# Autodesk Inventor assembly: BHSS
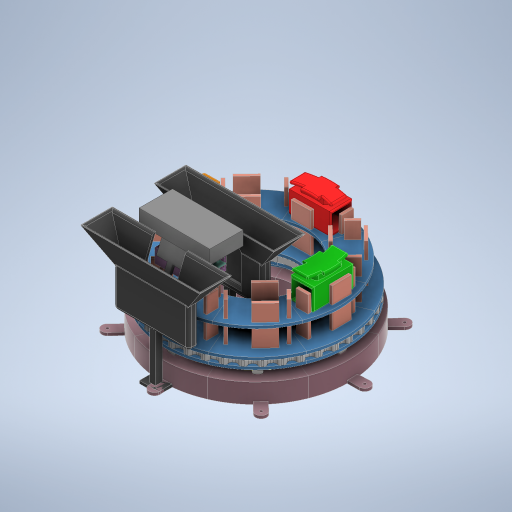
[picture p0: Inventor's stored thumbnail of the model, 512x512]
Saved by Autodesk Inventor 2023 (Build 270158000, 158)
## iProperties
Created: 2022-10-26
Part Number: BHSS
Document SubType Name: Assembly
Designer: cheng
Mass: 107138 g
Surface Area: 105016 cm^2
Volume: 89092.4 cm^3
Density: 1.20255 g/cm^3
Author: cheng
## Documents named in this file (11)
- C:\Users\mihal\Desktop\Current BHSS Design\Eighth Assembly\BHSS.iam
- C:\Users\mihal\Desktop\Current BHSS Design\Eighth Assembly\Battery Container.ipt
- C:\Users\mihal\Desktop\Current BHSS Design\Eighth Assembly\Box Base Plate.ipt
- C:\Users\mihal\Desktop\Current BHSS Design\Eighth Assembly\Carousel Fixed Track.ipt
- C:\Users\mihal\Desktop\Current BHSS Design\Eighth Assembly\drone model.ipt
- C:\Users\mihal\Desktop\Current BHSS Design\Eighth Assembly\Husky_3D_Model.ipt
- C:\Users\mihal\Desktop\Current BHSS Design\Eighth Assembly\Landing dock V2.ipt
- C:\Users\mihal\Desktop\Current BHSS Design\Eighth Assembly\Battery Cage Spring Plate.ipt
- C:\Users\mihal\Desktop\Current BHSS Design\Eighth Assembly\Inner Circle Landing Legs.ipt
- C:\Users\mihal\Desktop\Current BHSS Design\Eighth Assembly\Full Roller Carousel Assembly.iam
- C:\Users\mihal\Desktop\Current BHSS Design\Eighth Assembly\Battery Cage - Copy.ipt
## Components (25 placed, 13 different names)
1. Box Base Plate:1 — Mate:4, Mate:5, Mate:6, Mate:18, Mate:19, Mate:20, Mate:25, Flush:1, Mate:107, Mate:110, Mate:111, Mate:117, Mate:118
2. Carousel Fixed Track:1 — Mate:4, Mate:10, Mate:11
3. Carousel Fixed Track:2 — Mate:5, Mate:14, Mate:15, Mate:16, Mate:17, Mate:119
4. Carousel Fixed Track:3 — Mate:10, Mate:11, Mate:12, Mate:13, Mate:25, Rotating the Crousel
5. Carousel Fixed Track:4 — Mate:6, Mate:12, Mate:13, Mate:14, Mate:15, Mate:120
6. Carousel Fixed Track:5 — Mate:16, Mate:17, Mate:18, Mate:21, Mate:22
7. Carousel Fixed Track:6 — Mate:19, Mate:23, Mate:24, Mate:108, Mate:109
8. Carousel Fixed Track:7 — Mate:20, Mate:21, Mate:22, Mate:23, Mate:24
9. drone model:1 — Mate:145, Mate:146, Mate:147
10. Husky_3D_Model:1 — Flush:1
11. Red Battery — Side, Front, Bottom, Bat Wing Face to Cage Face, Mate:152
12. Carousel Fixed Track:8 — Mate:107, Mate:108, Mate:109
13. Landing dock V2:1 — Mate:110, Mate:111
14. Battery Cage Spring Plate:2 — Mate:148, Spring and top, Mate:152, Mate:153
15. Inner Circle Landing Legs:2 — Mate:117
16. Inner Circle Landing Legs:4 — Mate:118
17. Full Roller Carousel Assembly:1 [sub-assembly] — Mate:119, Mate:120, Side, Front, Mate:123, Mate:124, Mate:125, Mate:126, Mate:127, Mate:128, Mate:129, Mate:130, Mate:131, Mate:132, Mate:133, Mate:134, Mate:135, Mate:136, Mate:137, Mate:138, Mate:139, Mate:140, Mate:141, Mate:142, Bottom, Mate:144, Rotating the Crousel
18. Battery Container:20 — Mate:127, Mate:128, Mate:140
19. Battery Container:21 — Mate:131, Mate:132, Mate:138
20. Green Battery — Mate:125, Mate:126, Mate:141, Mate:153
21. Battery Container:23 — Mate:129, Mate:130, Mate:139
22. Orange Battery — Mate:133, Mate:134, Mate:137
23. Battery Container:25 — Mate:135, Mate:136, Mate:144
24. Battery Container:26 — Mate:123, Mate:124, Mate:142
25. Battery Cage - Copy:1 — Mate:145, Mate:146, Mate:147, Mate:148, Spring and top, Bat Wing Face to Cage Face
## Relationships (62: Mate 60, Flush 1, Angle 1)
- Mate:4: Box Base Plate:1 ↔ Carousel Fixed Track:1
- Mate:5: Box Base Plate:1 ↔ Carousel Fixed Track:2
- Mate:6: Box Base Plate:1 ↔ Carousel Fixed Track:4
- Mate:10: Carousel Fixed Track:1 ↔ Carousel Fixed Track:3
- Mate:11: Carousel Fixed Track:1 ↔ Carousel Fixed Track:3
- Mate:12: Carousel Fixed Track:3 ↔ Carousel Fixed Track:4
- Mate:13: Carousel Fixed Track:3 ↔ Carousel Fixed Track:4
- Mate:14: Carousel Fixed Track:2 ↔ Carousel Fixed Track:4
- Mate:15: Carousel Fixed Track:2 ↔ Carousel Fixed Track:4
- Mate:16: Carousel Fixed Track:2 ↔ Carousel Fixed Track:5
- Mate:17: Carousel Fixed Track:2 ↔ Carousel Fixed Track:5
- Mate:18: Box Base Plate:1 ↔ Carousel Fixed Track:5
- Mate:19: Box Base Plate:1 ↔ Carousel Fixed Track:6
- Mate:20: Box Base Plate:1 ↔ Carousel Fixed Track:7
- Mate:21: Carousel Fixed Track:5 ↔ Carousel Fixed Track:7
- Mate:22: Carousel Fixed Track:5 ↔ Carousel Fixed Track:7
- Mate:23: Carousel Fixed Track:6 ↔ Carousel Fixed Track:7
- Mate:24: Carousel Fixed Track:6 ↔ Carousel Fixed Track:7
- Mate:25: Box Base Plate:1 ↔ Carousel Fixed Track:3
- Flush:1: Box Base Plate:1 ↔ Husky_3D_Model:1
- Mate:107: Box Base Plate:1 ↔ Carousel Fixed Track:8
- Mate:108: Carousel Fixed Track:6 ↔ Carousel Fixed Track:8
- Mate:109: Carousel Fixed Track:6 ↔ Carousel Fixed Track:8
- Mate:110: Box Base Plate:1 ↔ Landing dock V2:1
- Mate:111: Box Base Plate:1 ↔ Landing dock V2:1
- Mate:117: Box Base Plate:1 ↔ Inner Circle Landing Legs:2
- Mate:118: Box Base Plate:1 ↔ Inner Circle Landing Legs:4
- Mate:119: Carousel Fixed Track:2 ↔ Full Roller Carousel Assembly:1
- Mate:120: Carousel Fixed Track:4 ↔ Full Roller Carousel Assembly:1
- Side [Mate]: Red Battery ↔ Full Roller Carousel Assembly:1
- Front [Mate]: Red Battery ↔ Full Roller Carousel Assembly:1
- Mate:123: Full Roller Carousel Assembly:1 ↔ Battery Container:26
- Mate:124: Full Roller Carousel Assembly:1 ↔ Battery Container:26
- Mate:125: Full Roller Carousel Assembly:1 ↔ Green Battery
- Mate:126: Full Roller Carousel Assembly:1 ↔ Green Battery
- Mate:127: Full Roller Carousel Assembly:1 ↔ Battery Container:20
- Mate:128: Full Roller Carousel Assembly:1 ↔ Battery Container:20
- Mate:129: Full Roller Carousel Assembly:1 ↔ Battery Container:23
- Mate:130: Full Roller Carousel Assembly:1 ↔ Battery Container:23
- Mate:131: Full Roller Carousel Assembly:1 ↔ Battery Container:21
- Mate:132: Full Roller Carousel Assembly:1 ↔ Battery Container:21
- Mate:133: Full Roller Carousel Assembly:1 ↔ Orange Battery
- Mate:134: Full Roller Carousel Assembly:1 ↔ Orange Battery
- Mate:135: Full Roller Carousel Assembly:1 ↔ Battery Container:25
- Mate:136: Full Roller Carousel Assembly:1 ↔ Battery Container:25
- Mate:137: Full Roller Carousel Assembly:1 ↔ Orange Battery
- Mate:138: Full Roller Carousel Assembly:1 ↔ Battery Container:21
- Mate:139: Full Roller Carousel Assembly:1 ↔ Battery Container:23
- Mate:140: Full Roller Carousel Assembly:1 ↔ Battery Container:20
- Mate:141: Full Roller Carousel Assembly:1 ↔ Green Battery
- Mate:142: Full Roller Carousel Assembly:1 ↔ Battery Container:26
- Bottom [Mate]: Red Battery ↔ Full Roller Carousel Assembly:1
- Mate:144: Full Roller Carousel Assembly:1 ↔ Battery Container:25
- Rotating the Crousel [Angle] (270 deg): Carousel Fixed Track:3 ↔ Full Roller Carousel Assembly:1
- Mate:145: drone model:1 ↔ Battery Cage - Copy:1
- Mate:146: drone model:1 ↔ Battery Cage - Copy:1
- Mate:147: drone model:1 ↔ Battery Cage - Copy:1
- Mate:148: Battery Cage Spring Plate:2 ↔ Battery Cage - Copy:1
- Spring and top [Mate] (-10 mm): Battery Cage Spring Plate:2 ↔ Battery Cage - Copy:1
- Bat Wing Face to Cage Face [Mate]: Red Battery ↔ Battery Cage - Copy:1
- Mate:152: Red Battery ↔ Battery Cage Spring Plate:2
- Mate:153: Battery Cage Spring Plate:2 ↔ Green Battery
